# Autodesk Inventor assembly: wheel_with_mounts_right
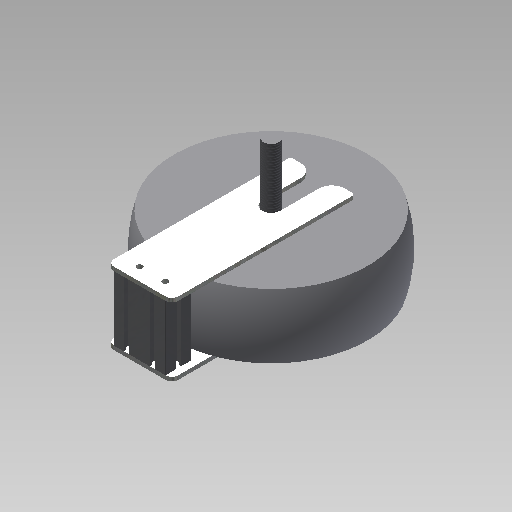
[picture p0: Inventor's stored thumbnail of the model, 512x512]
Saved by Autodesk Inventor 2021.2 (Build 252289000, 289)
## iProperties
Created: 2021-05-27
Part Number: wheel_with_mounts_right
Document SubType Name: Assembly
Designer: gisen
Author: gisen
## Documents named in this file (4)
- C:\Users\gisen\workspace\beetle_inventor_model\suspension\wheel_with_mounts_right.iam
- C:\Users\gisen\workspace\beetle_inventor_model\suspension\6inch_wheel_right.ipt
- C:\Users\gisen\workspace\beetle_inventor_model\suspension\wheel_mount_right.ipt
- C:\Users\gisen\workspace\beetle_inventor_model\suspension\AFS-2040-4-50_right.ipt
## Components (4 placed, 1 different names)
1. Part1:1 — メイト:2, メイト:1, メイト:12, フラッシュ:10, フラッシュ:3, メイト:3, フラッシュ:2
2. Part1:2 — メイト:12, フラッシュ:12, フラッシュ:10, フラッシュ:3, メイト:3, フラッシュ:11, メイト:4
3. Part1:3 — メイト:11
4. Part1:4 — フラッシュ:11, フラッシュ:2, メイト:4, メイト:11
## Relationships (11: Mate 9, Flush 2)
- メイト:2 [Mate]: Part1:1
- メイト:1 [Mate]: Part1:1
- メイト:12 [Mate]: Part1:1 ↔ Part1:2
- フラッシュ:12 [Mate]: Part1:2
- フラッシュ:10 [Mate]: Part1:1 ↔ Part1:2
- フラッシュ:3 [Mate]: Part1:1 ↔ Part1:2
- メイト:3 [Mate]: Part1:1 ↔ Part1:2
- フラッシュ:11 [Flush]: Part1:2 ↔ Part1:4
- フラッシュ:2 [Flush]: Part1:1 ↔ Part1:4
- メイト:4 [Mate]: Part1:2 ↔ Part1:4
- メイト:11 [Mate]: Part1:3 ↔ Part1:4
